# Autodesk Inventor assembly: Rack_truncated
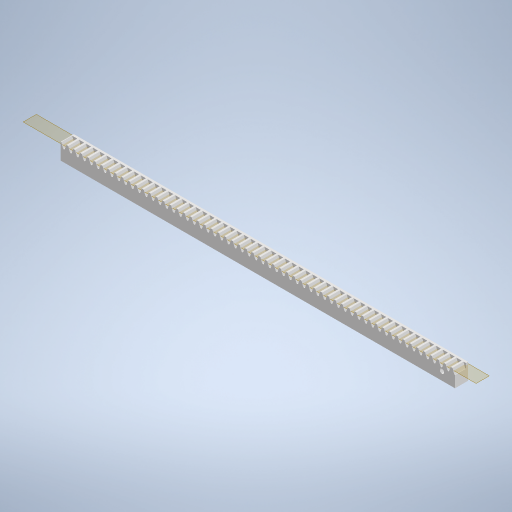
[picture p0: Inventor's stored thumbnail of the model, 512x512]
Saved by Autodesk Inventor 2023 (Build 270158000, 158)
## iProperties
Created: 2022-08-25
Part Number: Rack_truncated
Document SubType Name: Assembly
Designer: matte
Author: matte
## Documents named in this file (2)
- C:\Users\matte\Documents\GitHub\MDM-CyberOrto-CAD\Rack_Pinion\Rack_truncated.iam
- C:\Users\matte\Documents\GitHub\MDM-CyberOrto-CAD\Rack_Pinion\Rack.ipt
## Components (1 placed, 1 different names)
1. Rack:1
## Named parameters: len = 361 mm
